# Autodesk Inventor assembly: RollerIntake2.0
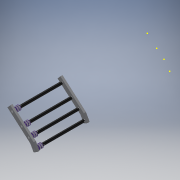
[picture p0: Inventor's stored thumbnail of the model, 180x180]
Saved by Autodesk Inventor 2018.3 (Build 223284000, 284)
## iProperties
Created: 2020-02-03
Part Number: RollerIntake2.0
Document SubType Name: Assembly
Designer: 22turnmaxw
Author: 22turnmaxw
## Documents named in this file (3)
- C:\Users\22barlalex\Documents\GrabCAD\Infinite Recharge 2020\Build season\ARM_023_Intake.iam
- C:\Users\22barlalex\Documents\GrabCAD\Infinite Recharge 2020\Build season\ARM_024_IntakeFrame.ipt
- C:\Users\22barlalex\Documents\GrabCAD\Infinite Recharge 2020\Build season\ARM_013_RollerBar.iam
## Components (6 placed, 2 different names)
1. ARM_024_IntakeFrame:1 — Flush:1, Flush:2, Mate:3
2. ARM_024_IntakeFrame:2 — Flush:1, Flush:2, Mate:1, Mate:2, Mate:4, Mate:5, Mate:6, Mate:7, Mate:8, Mate:9
3. ARM_013_RollerBar:1 [sub-assembly] — Mate:1, Mate:2, Mate:3
4. ARM_013_RollerBar:2 [sub-assembly] — Mate:4, Mate:5
5. ARM_013_RollerBar:3 [sub-assembly] — Mate:6, Mate:7
6. ARM_013_RollerBar:4 [sub-assembly] — Mate:8, Mate:9
## Relationships (11: Mate 9, Flush 2)
- Flush:1: ARM_024_IntakeFrame:1 ↔ ARM_024_IntakeFrame:2
- Flush:2: ARM_024_IntakeFrame:1 ↔ ARM_024_IntakeFrame:2
- Mate:1: ARM_024_IntakeFrame:2 ↔ ARM_013_RollerBar:1
- Mate:2: ARM_024_IntakeFrame:2 ↔ ARM_013_RollerBar:1
- Mate:3: ARM_024_IntakeFrame:1 ↔ ARM_013_RollerBar:1
- Mate:4: ARM_024_IntakeFrame:2 ↔ ARM_013_RollerBar:2
- Mate:5: ARM_024_IntakeFrame:2 ↔ ARM_013_RollerBar:2
- Mate:6: ARM_024_IntakeFrame:2 ↔ ARM_013_RollerBar:3
- Mate:7: ARM_024_IntakeFrame:2 ↔ ARM_013_RollerBar:3
- Mate:8: ARM_024_IntakeFrame:2 ↔ ARM_013_RollerBar:4
- Mate:9: ARM_024_IntakeFrame:2 ↔ ARM_013_RollerBar:4
